# Autodesk Inventor assembly: Finger_Baugruppe
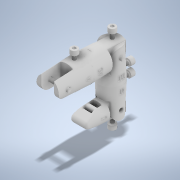
[picture p0: Inventor's stored thumbnail of the model, 180x180]
Saved by Autodesk Inventor 2021 (Build 250183000, 183)
## iProperties
Created: 2021-05-01
Part Number: Finger_Baugruppe
Document SubType Name: Assembly
Designer: Maxim
Author: Maxim
## Documents named in this file (9)
- D:\MEDS Studium\4. Semester\Informatik IV\Bionic Hand Version 1.1\Finger_Baugruppe.iam
- D:\MEDS Studium\4. Semester\Informatik IV\Bionic Hand Version 1.1\Fingerteil_3.ipt
- D:\MEDS Studium\4. Semester\Informatik IV\Bionic Hand Version 1.1\Fingerteil_4.ipt
- D:\MEDS Studium\4. Semester\Informatik IV\Bionic Hand Version 1.1\Fingerteil_1.ipt
- D:\MEDS Studium\4. Semester\Informatik IV\Bionic Hand Version 1.1\Fingerteil_2.ipt
- D:\MEDS Studium\4. Semester\Informatik IV\Bionic Hand Version 1.1\din_en_iso_4762_m3x10.ipt
- D:\MEDS Studium\4. Semester\Informatik IV\Bionic Hand Version 1.1\stift_iso_2338-3m6x20-a1.ipt
- D:\MEDS Studium\4. Semester\Informatik IV\Bionic Hand Version 1.1\Fingerteil_5.ipt
- D:\MEDS Studium\4. Semester\Informatik IV\Bionic Hand Version 1.1\din_en_iso_4762_m3x8.ipt
## Components (13 placed, 8 different names)
1. Fingerteil_1:1 — Fluchtend:3, Passend:11, Passend:12, Fluchtend:7, Zylindrisch:1
2. Fingerteil_2:1 — Passend:39, Passend:40, Fluchtend:6, Passend:45, Passend:46, Passend:48, Zylindrisch:1
3. Fingerteil_3:1 — Passend:38, Passend:39, Passend:40, Fluchtend:6, Passend:43, Passend:44, Passend:47, Zylindrisch:2
4. Fingerteil_4:1 — Passend:35, Fluchtend:5, Passend:36, Passend:41, Passend:42, Zylindrisch:2
5. Fingerteil_5:1 — Passend:29, Passend:30, Passend:31, Passend:32, Passend:33, Fluchtend:4, Passend:34, Passend:35, Fluchtend:5, Passend:36
6. din_en_iso_4762_m3x8:1 — Passend:45, Passend:46
7. din_en_iso_4762_m3x8:2 — Passend:43, Passend:44
8. din_en_iso_4762_m3x10:1 — Passend:11, Passend:12
9. din_en_iso_4762_m3x10:4 — Passend:41, Passend:42
10. din_en_iso_4762_m3x10:5 — Passend:29, Passend:30
11. stift_iso_2338-3m6x20-a1:1 — Passend:31, Passend:32
12. stift_iso_2338-3m6x20-a1:2 — Fluchtend:9, Passend:48
13. stift_iso_2338-3m6x20-a1:3 — Fluchtend:8, Passend:47
## Relationships (30: Mate 21, Flush 7, CylindricalJoint 2)
- Fluchtend:3 [Flush]: Fingerteil_1:1
- Passend:11 [Mate]: Fingerteil_1:1 ↔ din_en_iso_4762_m3x10:1
- Passend:12 [Mate]: Fingerteil_1:1 ↔ din_en_iso_4762_m3x10:1
- Passend:29 [Mate]: Fingerteil_5:1 ↔ din_en_iso_4762_m3x10:5
- Passend:30 [Mate]: Fingerteil_5:1 ↔ din_en_iso_4762_m3x10:5
- Passend:31 [Mate]: Fingerteil_5:1 ↔ stift_iso_2338-3m6x20-a1:1
- Passend:32 [Mate] (-10 mm): Fingerteil_5:1 ↔ stift_iso_2338-3m6x20-a1:1
- Passend:33 [Mate]: Fingerteil_5:1
- Fluchtend:4 [Flush]: Fingerteil_5:1
- Passend:34 [Mate]: Fingerteil_5:1
- Passend:35 [Mate]: Fingerteil_4:1 ↔ Fingerteil_5:1
- Fluchtend:5 [Flush]: Fingerteil_4:1 ↔ Fingerteil_5:1
- Passend:36 [Mate]: Fingerteil_4:1 ↔ Fingerteil_5:1
- Passend:38 [Mate]: Fingerteil_3:1
- Passend:39 [Mate]: Fingerteil_2:1 ↔ Fingerteil_3:1
- Passend:40 [Mate]: Fingerteil_2:1 ↔ Fingerteil_3:1
- Fluchtend:6 [Flush]: Fingerteil_2:1 ↔ Fingerteil_3:1
- Fluchtend:7 [Flush]: Fingerteil_1:1
- Passend:41 [Mate]: Fingerteil_4:1 ↔ din_en_iso_4762_m3x10:4
- Passend:42 [Mate]: Fingerteil_4:1 ↔ din_en_iso_4762_m3x10:4
- Passend:43 [Mate]: Fingerteil_3:1 ↔ din_en_iso_4762_m3x8:2
- Passend:44 [Mate]: Fingerteil_3:1 ↔ din_en_iso_4762_m3x8:2
- Passend:45 [Mate]: Fingerteil_2:1 ↔ din_en_iso_4762_m3x8:1
- Passend:46 [Mate]: Fingerteil_2:1 ↔ din_en_iso_4762_m3x8:1
- Fluchtend:8 [Flush] (-10 mm): stift_iso_2338-3m6x20-a1:3
- Passend:47 [Mate]: Fingerteil_3:1 ↔ stift_iso_2338-3m6x20-a1:3
- Fluchtend:9 [Flush] (-10 mm): stift_iso_2338-3m6x20-a1:2
- Passend:48 [Mate]: Fingerteil_2:1 ↔ stift_iso_2338-3m6x20-a1:2
- Zylindrisch:1 [CylindricalJoint]: Fingerteil_1:1 ↔ Fingerteil_2:1
- Zylindrisch:2 [CylindricalJoint]: Fingerteil_3:1 ↔ Fingerteil_4:1
